# Autodesk Inventor assembly: rpiWCase
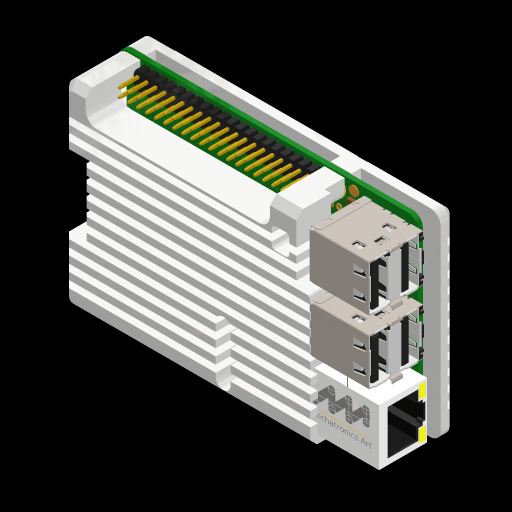
[picture p0: Inventor's stored thumbnail of the model, 512x512]
Saved by Autodesk Inventor 2023 (Build 270158000, 158)
## iProperties
Created: 2022-07-18
Part Number: rpiWCase
Document SubType Name: Assembly
Designer: Fuzzyfish
Author: Fuzzyfish
## Documents named in this file (4)
- C:\Users\Fuzzyfish\Documents\Inventor\finalBox\rpiWCase.iam
- C:\Users\Fuzzyfish\Documents\Inventor\finalBox\raspberry-pi-3-model-b-reference-design-solidworks-cad-rpi-raspberrypi-raspberry-pi-1.snapshot.83 (1)\Exported Versions\STEP\Raspberry Pi 3.iam
- C:\Users\Fuzzyfish\Documents\Inventor\finalBox\raspberry-pi-3-model-b-reference-design-solidworks-cad-rpi-raspberrypi-raspberry-pi-1.snapshot.83 (1)\Exported Versions\STEP\heatsink-bottom.ipt
- C:\Users\Fuzzyfish\Documents\Inventor\finalBox\raspberry-pi-3-model-b-reference-design-solidworks-cad-rpi-raspberrypi-raspberry-pi-1.snapshot.83 (1)\Exported Versions\STEP\heatsink-top.ipt
## Components (3 placed, 3 different names)
1. Raspberry Pi 3:1 [sub-assembly] — Mate:1, Mate:2, Mate:3, Mate:4, Mate:5, Mate:6
2. heatsink-bottom:1 — Mate:1, Mate:2, Mate:3
3. heatsink-top:1 — Mate:4, Mate:5, Mate:6
## Relationships (6: Mate 6)
- Mate:1: Raspberry Pi 3:1 ↔ heatsink-bottom:1
- Mate:2: Raspberry Pi 3:1 ↔ heatsink-bottom:1
- Mate:3: Raspberry Pi 3:1 ↔ heatsink-bottom:1
- Mate:4: Raspberry Pi 3:1 ↔ heatsink-top:1
- Mate:5: Raspberry Pi 3:1 ↔ heatsink-top:1
- Mate:6: Raspberry Pi 3:1 ↔ heatsink-top:1
